# Autodesk Inventor assembly: Assembly1
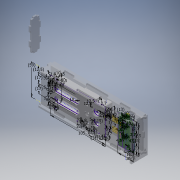
[picture p0: Inventor's stored thumbnail of the model, 180x180]
Saved by Autodesk Inventor 2016 (Build 200138000, 138)
## iProperties
Created: 2015-06-16
Part Number: Assembly1
Document SubType Name: Assembly
Designer: Openlab
Author: Openlab
## Documents named in this file (14)
- D:\Alexey\HS-Spectrophotometer\parts\Assembly1.iam
- D:\Alexey\HS-Spectrophotometer\parts\Bottom_V3.ipt
- D:\Alexey\HS-Spectrophotometer\parts\Led_Board_V1.ipt
- D:\Alexey\HS-Spectrophotometer\parts\Sensor_Board_dummy.ipt
- D:\Alexey\HS-Spectrophotometer\parts\Top_V4.ipt
- D:\Alexey\HS-Spectrophotometer\parts\Top_plate2.ipt
- D:\Alexey\HS-Spectrophotometer\parts\Large_retainer.ipt
- D:\Alexey\HS-Spectrophotometer\parts\Bottom_plate2.ipt
- D:\Alexey\HS-Spectrophotometer\parts\Left_wall.ipt
- D:\Alexey\HS-Spectrophotometer\parts\Right_wall.ipt
- D:\Alexey\HS-Spectrophotometer\parts\Cuvette_retainer2.ipt
- D:\Alexey\HS-Spectrophotometer\parts\Motherboard_assembly.iam
- D:\Alexey\HS-Spectrophotometer\parts\Back_Wall.ipt
- D:\Alexey\HS-Spectrophotometer\parts\Front_wall.ipt
## Components (15 placed, 13 different names)
1. Bottom_V3:1 — Mate:1, Mate:4, Mate:7, Mate:10, Mate:11, Mate:12, Mate:13, Mate:14, Mate:15, Mate:16, Mate:52, Mate:53, Mate:54, Mate:64, Mate:65, Mate:66
2. Led_Board_V1:1 — Mate:4, Mate:13, Mate:14
3. Sensor_Board_dummy:1 — Mate:7, Mate:15, Mate:16
4. Top_V4:1 — Mate:1, Mate:52, Mate:53, Mate:54
5. Top_plate2:1 — Mate:71, Mate:72, Mate:76, Mate:77, Mate:78, Mate:79, Mate:80
6. Large_retainer:1
7. Large_retainer:2
8. Bottom_plate2:1 — Mate:56, Mate:57, Mate:61, Mate:64, Mate:65, Mate:66, Mate:73, Mate:75
9. Left_wall:1 — Mate:56, Mate:57, Mate:67, Mate:68, Mate:71, Mate:74, Mate:75, Mate:76, Mate:77, Flush:1, Flush:2, Mate:81
10. Right_wall:1 — Mate:61, Mate:72, Mate:73
11. Cuvette_retainer2:1 — Mate:10, Mate:11, Mate:12
12. Motherboard_assembly:1 [sub-assembly] — Mate:67, Mate:68, Mate:74
13. Back_Wall:1
14. Front_wall:1 — Flush:1, Flush:2, Mate:81
15. Left_wall:2 — Mate:78, Mate:79, Mate:80
## Relationships (34: Mate 32, Flush 2)
- Mate:1: Bottom_V3:1 ↔ Top_V4:1
- Mate:4: Bottom_V3:1 ↔ Led_Board_V1:1
- Mate:7: Bottom_V3:1 ↔ Sensor_Board_dummy:1
- Mate:10: Bottom_V3:1 ↔ Cuvette_retainer2:1
- Mate:11: Bottom_V3:1 ↔ Cuvette_retainer2:1
- Mate:12: Bottom_V3:1 ↔ Cuvette_retainer2:1
- Mate:13: Bottom_V3:1 ↔ Led_Board_V1:1
- Mate:14: Bottom_V3:1 ↔ Led_Board_V1:1
- Mate:15: Bottom_V3:1 ↔ Sensor_Board_dummy:1
- Mate:16: Bottom_V3:1 ↔ Sensor_Board_dummy:1
- Mate:52: Bottom_V3:1 ↔ Top_V4:1
- Mate:53: Bottom_V3:1 ↔ Top_V4:1
- Mate:54: Bottom_V3:1 ↔ Top_V4:1
- Mate:56: Bottom_plate2:1 ↔ Left_wall:1
- Mate:57: Bottom_plate2:1 ↔ Left_wall:1
- Mate:61: Bottom_plate2:1 ↔ Right_wall:1
- Mate:64: Bottom_V3:1 ↔ Bottom_plate2:1
- Mate:65: Bottom_V3:1 ↔ Bottom_plate2:1
- Mate:66: Bottom_V3:1 ↔ Bottom_plate2:1
- Mate:67: Left_wall:1 ↔ Motherboard_assembly:1
- Mate:68: Left_wall:1 ↔ Motherboard_assembly:1
- Mate:71: Top_plate2:1 ↔ Left_wall:1
- Mate:72: Top_plate2:1 ↔ Right_wall:1
- Mate:73: Bottom_plate2:1 ↔ Right_wall:1
- Mate:74: Left_wall:1 ↔ Motherboard_assembly:1
- Mate:75: Bottom_plate2:1 ↔ Left_wall:1
- Mate:76: Top_plate2:1 ↔ Left_wall:1
- Mate:77: Top_plate2:1 ↔ Left_wall:1
- Flush:1: Left_wall:1 ↔ Front_wall:1
- Mate:78: Top_plate2:1 ↔ Left_wall:2
- Mate:79: Top_plate2:1 ↔ Left_wall:2
- Mate:80: Top_plate2:1 ↔ Left_wall:2
- Flush:2: Left_wall:1 ↔ Front_wall:1
- Mate:81: Left_wall:1 ↔ Front_wall:1
